# Autodesk Inventor assembly: LagSamlet
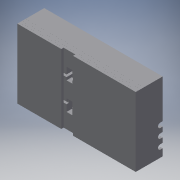
[picture p0: Inventor's stored thumbnail of the model, 180x180]
Saved by Autodesk Inventor 2016 (Build 200138000, 138)
## iProperties
Created: 2016-12-11
Part Number: LagSamlet
Document SubType Name: Assembly
Designer: Simon
Author: Simon
## Documents named in this file (6)
- E:\OneDrive\HTX\Teknologi\YE\LagSamlet.iam
- E:\OneDrive\HTX\Teknologi\YE\Lag1.ipt
- E:\OneDrive\HTX\Teknologi\YE\Lag2.ipt
- E:\OneDrive\HTX\Teknologi\YE\Lag 3.ipt
- E:\OneDrive\HTX\Teknologi\YE\Lag4.ipt
- E:\OneDrive\HTX\Teknologi\YE\Lag5.ipt
## Components (5 placed, 5 different names)
1. Lag1:1 — Mate:1, Mate:2, Mate:7, Mate:8
2. Lag2:1 — Mate:1, Mate:2, Mate:3, Mate:4, Mate:7, Mate:8
3. Lag 3:1 — Mate:3, Mate:4, Mate:5, Mate:6, Mate:9, Mate:10, Mate:11, Mate:12
4. Lag4:1 — Mate:5, Mate:6, Mate:9, Mate:10, Mate:11, Mate:12, Mate:13, Mate:14
5. Lag5:1 — Mate:13, Mate:14
## Relationships (14: Mate 14)
- Mate:1: Lag1:1 ↔ Lag2:1
- Mate:2: Lag1:1 ↔ Lag2:1
- Mate:3: Lag2:1 ↔ Lag 3:1
- Mate:4: Lag2:1 ↔ Lag 3:1
- Mate:5: Lag 3:1 ↔ Lag4:1
- Mate:6: Lag 3:1 ↔ Lag4:1
- Mate:7: Lag1:1 ↔ Lag2:1
- Mate:8: Lag1:1 ↔ Lag2:1
- Mate:9: Lag 3:1 ↔ Lag4:1
- Mate:10: Lag 3:1 ↔ Lag4:1
- Mate:11: Lag 3:1 ↔ Lag4:1
- Mate:12: Lag 3:1 ↔ Lag4:1
- Mate:13: Lag4:1 ↔ Lag5:1
- Mate:14: Lag4:1 ↔ Lag5:1
